# Autodesk Inventor assembly: extension arm middle
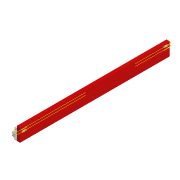
[picture p0: Inventor's stored thumbnail of the model, 180x180]
Saved by Autodesk Inventor 2020 (Build 240168000, 168)
## iProperties
Created: 2019-12-12
Part Number: extension arm middle
Document SubType Name: Assembly
Designer: ball
Author: ball
## Documents named in this file (4)
- C:\FTC\FTC8863CAD\2019 Robot\Delivery\extension arm\extension arm middle.iam
- C:\FTC\FTC8863CAD\Misumi\SAR340\SAR340 offset 10 mm.iam
- C:\FTC\FTC8863CAD\2019 Robot\Delivery\extension arm\couple extension arm motor middle + pulleys.iam
- C:\FTC\FTC8863CAD\2019 Robot\Delivery\extension arm\coupler extention arm collector middle + pulleys.iam
## Components (3 placed, 3 different names)
1. SAR340 offset 10 mm:1 [sub-assembly] — Mate:6, Mate:7, Mate:8, Mate:9, Mate:10, Flush:1
2. couple extension arm motor middle + pulleys:1 [sub-assembly] — Mate:6, Mate:7, Mate:8
3. coupler extention arm collector middle + pulleys:1 [sub-assembly] — Mate:9, Mate:10, Flush:1
## Relationships (6: Mate 5, Flush 1)
- Mate:6: SAR340 offset 10 mm:1 ↔ couple extension arm motor middle + pulleys:1
- Mate:7: SAR340 offset 10 mm:1 ↔ couple extension arm motor middle + pulleys:1
- Mate:8: SAR340 offset 10 mm:1 ↔ couple extension arm motor middle + pulleys:1
- Mate:9: SAR340 offset 10 mm:1 ↔ coupler extention arm collector middle + pulleys:1
- Mate:10: SAR340 offset 10 mm:1 ↔ coupler extention arm collector middle + pulleys:1
- Flush:1: SAR340 offset 10 mm:1 ↔ coupler extention arm collector middle + pulleys:1
